# Autodesk Inventor assembly: lab view of cryostat
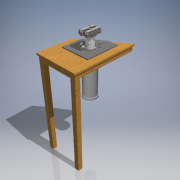
[picture p0: Inventor's stored thumbnail of the model, 180x180]
Saved by Autodesk Inventor 2018 (Build 220112000, 112)
## iProperties
Created: 2018-10-18
Part Number: lab view of cryostat
Document SubType Name: Assembly
Designer: freyja
Author: freyja
## Documents named in this file (5)
- C:\Users\freyja\Documents\Cryorefrigerator\CAD\lab view of cryostat.iam
- C:\Users\freyja\Documents\Cryorefrigerator\CAD\table.ipt
- C:\Users\freyja\Documents\Cryorefrigerator\CAD\mini Cryostat FOOT3.iam
- C:\Users\freyja\Documents\Cryorefrigerator\CAD\table reinforcement.ipt
- C:\Users\freyja\Documents\Cryorefrigerator\CAD\pulley.iam
## Components (6 placed, 4 different names)
1. table:1 — Mate:1, Angle:1, Mate:2, Mate:5, Mate:6, Mate:16, Angle:2
2. mini Cryostat FOOT3:1 [sub-assembly] — Mate:1, Angle:1, Mate:2, Mate:4, Mate:7, Mate:8, Mate:9
3. table reinforcement:1 — Mate:4, Mate:5, Mate:8, Mate:10, Mate:14, Mate:15
4. table reinforcement:2 — Mate:6, Mate:7, Mate:9, Mate:11, Mate:12, Mate:13
5. pulley:1 [sub-assembly] — Mate:11, Mate:12, Mate:13
6. pulley:2 [sub-assembly] — Mate:10, Mate:14, Mate:15
## Relationships (17: Mate 15, Angle 2)
- Mate:1: table:1 ↔ mini Cryostat FOOT3:1
- Angle:1 (0 deg): table:1 ↔ mini Cryostat FOOT3:1
- Mate:2: table:1 ↔ mini Cryostat FOOT3:1
- Mate:4: mini Cryostat FOOT3:1 ↔ table reinforcement:1
- Mate:5: table:1 ↔ table reinforcement:1
- Mate:6: table:1 ↔ table reinforcement:2
- Mate:7: mini Cryostat FOOT3:1 ↔ table reinforcement:2
- Mate:8: mini Cryostat FOOT3:1 ↔ table reinforcement:1
- Mate:9: mini Cryostat FOOT3:1 ↔ table reinforcement:2
- Mate:10: table reinforcement:1 ↔ pulley:2
- Mate:11: table reinforcement:2 ↔ pulley:1
- Mate:12: table reinforcement:2 ↔ pulley:1
- Mate:13: table reinforcement:2 ↔ pulley:1
- Mate:14: table reinforcement:1 ↔ pulley:2
- Mate:15: table reinforcement:1 ↔ pulley:2
- Mate:16: table:1
- Angle:2 (55 deg): table:1
